# Autodesk Inventor assembly: Prototype_LaserNavegationSystem
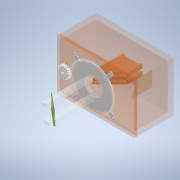
[picture p0: Inventor's stored thumbnail of the model, 180x180]
Saved by Autodesk Inventor 2022.2 (Build 262287010, 287A)
## iProperties
Created: 2022-03-17
Part Number: Prototype_LaserNavegationSystem
Document SubType Name: Assembly
Designer: mabel
Author: mabel
## Documents named in this file (10)
- D:\GitHub\laser-nav\Mechanics\Prototype_LaserNavegationSystem.iam
- C:\Users\mabel\OneDrive\Documentos\Inventor\LaserNavigationSystem\Cambio\EngraneN18.ipt
- C:\Users\mabel\OneDrive\Documentos\Inventor\LaserNavigationSystem\Cambio\EngraneN72.ipt
- C:\Users\mabel\OneDrive\Documentos\Inventor\LaserNavigationSystem\Cambio\Tapa.ipt
- C:\Users\mabel\OneDrive\Documentos\Inventor\LaserNavigationSystem\Cambio\EjeMotor.ipt
- C:\Users\mabel\OneDrive\Documentos\Inventor\LaserNavigationSystem\Cambio\CajaOscura.ipt
- C:\Users\mabel\OneDrive\Documentos\Inventor\LaserNavigationSystem\Base-BeamSplitter.ipt
- C:\Users\mabel\OneDrive\Documentos\Inventor\LaserNavigationSystem\BeamSplitter.ipt
- C:\Users\mabel\OneDrive\Documentos\Inventor\LaserNavigationSystem\Cambio\SoportaEspejo.ipt
- C:\Users\mabel\OneDrive\Documentos\Inventor\LaserNavigationSystem\Cambio\Anillo.ipt
## Components (10 placed, 9 different names)
1. Engranaje rectoN18:1 — Coincidencia:4, Coincidencia:11, Coincidencia:17
2. Tapa:1 — Coincidencia:4, Nivelación:2, Nivelación:3, Coincidencia:11, Coincidencia:12, Coincidencia:18, Coincidencia:19, Coincidencia:20, Coincidencia:21, Coincidencia:22, Coincidencia:23
3. CajaOscura:1 — Nivelación:2, Nivelación:3
4. Base-BeamSplitter:1 — Coincidencia:7
5. BeamSplitter:1 — Coincidencia:7
6. Engranaje rectoN72:1 — Coincidencia:12, Coincidencia:15, Coincidencia:16, Coincidencia:18, Coincidencia:23
7. SoportaEspejo:1 — Coincidencia:15, Coincidencia:16
8. EjeMotor:1 — Coincidencia:17
9. Anillo:1 — Coincidencia:19, Coincidencia:21
10. Anillo:2 — Coincidencia:20, Coincidencia:22
## Relationships (15: Mate 13, Flush 2)
- Coincidencia:4 [Mate]: Engranaje rectoN18:1 ↔ Tapa:1
- Nivelación:2 [Flush]: Tapa:1 ↔ CajaOscura:1
- Nivelación:3 [Flush]: Tapa:1 ↔ CajaOscura:1
- Coincidencia:7 [Mate]: Base-BeamSplitter:1 ↔ BeamSplitter:1
- Coincidencia:11 [Mate] (3 mm): Engranaje rectoN18:1 ↔ Tapa:1
- Coincidencia:12 [Mate]: Tapa:1 ↔ Engranaje rectoN72:1
- Coincidencia:15 [Mate]: Engranaje rectoN72:1 ↔ SoportaEspejo:1
- Coincidencia:16 [Mate]: Engranaje rectoN72:1 ↔ SoportaEspejo:1
- Coincidencia:17 [Mate]: Engranaje rectoN18:1 ↔ EjeMotor:1
- Coincidencia:18 [Mate]: Tapa:1 ↔ Engranaje rectoN72:1
- Coincidencia:19 [Mate]: Tapa:1 ↔ Anillo:1
- Coincidencia:20 [Mate]: Tapa:1 ↔ Anillo:2
- Coincidencia:21 [Mate]: Tapa:1 ↔ Anillo:1
- Coincidencia:22 [Mate]: Tapa:1 ↔ Anillo:2
- Coincidencia:23 [Mate]: Tapa:1 ↔ Engranaje rectoN72:1
